# Autodesk Inventor assembly: hodoscopeHolder
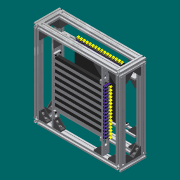
[picture p0: Inventor's stored thumbnail of the model, 180x180]
Saved by Autodesk Inventor 2016 (Build 200138000, 138)
## iProperties
Created: 2016-02-10
Part Number: hodoscopeHolder
Document SubType Name: Assembly
Designer: Sawaiz
Author: Sawaiz
## Documents named in this file (5)
- C:\Users\Sawaiz\OneDrive\projects\modularRICH\testMount\fingerHodoscope\hodoscopeHolder.iam
- C:\Users\Sawaiz\OneDrive\projects\modularRICH\testMount\fingerHodoscope\face.iam
- C:\Users\Sawaiz\OneDrive\projects\modularRICH\testMount\fingerHodoscope\hfs5-2020-HodoscopeSeperator.ipt
- C:\Users\Sawaiz\OneDrive\projects\modularRICH\testMount\frame\angleBracket.iam
- C:\Users\Sawaiz\OneDrive\projects\scintillatorPanel\4xStack.iam
## Components (24 placed, 4 different names)
1. face:1 [sub-assembly] — Flush:1, Flush:2, Symmetry:1, Symmetry:2, Symmetry:3, Flush:3, Flush:4, Flush:5, Flush:6, Mate:2, Mate:3, Flush:7, Flush:8, Flush:9, Flush:10, Flush:11, Flush:12, Flush:13, Flush:14, Flush:29, Mate:15, Mate:18, Mate:20, Flush:39, Mate:22, Mate:25, Flush:70, Mate:36, Flush:71, Mate:42
2. face:2 [sub-assembly] — Flush:1, Flush:2, Symmetry:1, Symmetry:2, Symmetry:3, Mate:1, Flush:15, Mate:23, Mate:26, Flush:53, Mate:34, Mate:37, Mate:38, Flush:72, Mate:45
3. hfs5-2020-HodoscopeSeperator:1 — Mate:1, Flush:3, Flush:12, Flush:13, Flush:14, Mate:35
4. hfs5-2020-HodoscopeSeperator:2 — Flush:4, Flush:9, Flush:10, Flush:11, Flush:15, Mate:27
5. hfs5-2020-HodoscopeSeperator:3 — Flush:6, Mate:2, Mate:3, Mate:39
6. hfs5-2020-HodoscopeSeperator:4 — Flush:5, Flush:7, Flush:8, Flush:38, Mate:24
7. angleBracket:1 [sub-assembly] — Flush:26, Mate:20, Flush:56
8. angleBracket:2 [sub-assembly] — Flush:26, Flush:27, Flush:30, Mate:15, Symmetry:6, Flush:56, Mate:40
9. angleBracket:3 [sub-assembly] — Flush:27, Flush:28, Flush:30, Symmetry:6, Flush:57, Mate:41
10. angleBracket:4 [sub-assembly] — Flush:28, Flush:29, Mate:18, Flush:57
11. angleBracket:5 [sub-assembly] — Flush:24, Flush:34, Flush:52, Flush:55, Mate:43
12. angleBracket:6 [sub-assembly] — Flush:23, Flush:24, Flush:32, Flush:50, Flush:51, Symmetry:4, Symmetry:5, Flush:54
13. angleBracket:7 [sub-assembly] — Flush:22, Flush:23, Flush:34, Flush:51, Flush:52, Symmetry:4, Flush:53, Mate:34, Flush:54, Mate:44
14. angleBracket:8 [sub-assembly] — Flush:22, Flush:32, Flush:50, Symmetry:5, Flush:55
15. angleBracket:9 [sub-assembly] — Flush:37, Flush:38, Flush:41, Mate:26, Mate:27
16. angleBracket:10 [sub-assembly] — Flush:36, Flush:37, Mate:22, Flush:40, Mate:24
17. angleBracket:11 [sub-assembly] — Flush:35, Flush:36, Flush:39, Mate:23, Flush:40
18. angleBracket:12 [sub-assembly] — Flush:35, Flush:41, Mate:25
19. 4xStack:1 [sub-assembly] — Mate:40, Mate:41, Flush:71, Mate:42
20. 4xStack:2 [sub-assembly] — Mate:43, Mate:44, Flush:72, Mate:45
21. angleBracket:13 [sub-assembly] — Flush:65, Flush:66, Flush:67, Flush:68, Mate:37
22. angleBracket:14 [sub-assembly] — Flush:63, Flush:64, Flush:68, Flush:69, Mate:39
23. angleBracket:15 [sub-assembly] — Flush:63, Flush:69, Mate:38
24. angleBracket:16 [sub-assembly] — Flush:64, Flush:65, Flush:66, Mate:35, Flush:67, Flush:70, Mate:36
## Relationships (85: Flush 55, Mate 24, Symmetry 6)
- Flush:1: face:1 ↔ face:2
- Flush:2: face:1 ↔ face:2
- Symmetry:1: face:1 ↔ face:2
- Symmetry:2: face:1 ↔ face:2
- Symmetry:3: face:1 ↔ face:2
- Mate:1: face:2 ↔ hfs5-2020-HodoscopeSeperator:1
- Flush:3: face:1 ↔ hfs5-2020-HodoscopeSeperator:1
- Flush:4: face:1 ↔ hfs5-2020-HodoscopeSeperator:2
- Flush:5: face:1 ↔ hfs5-2020-HodoscopeSeperator:4
- Flush:6: face:1 ↔ hfs5-2020-HodoscopeSeperator:3
- Mate:2: face:1 ↔ hfs5-2020-HodoscopeSeperator:3
- Mate:3: face:1 ↔ hfs5-2020-HodoscopeSeperator:3
- Flush:7: face:1 ↔ hfs5-2020-HodoscopeSeperator:4
- Flush:8: face:1 ↔ hfs5-2020-HodoscopeSeperator:4
- Flush:9: face:1 ↔ hfs5-2020-HodoscopeSeperator:2
- Flush:10: face:1 ↔ hfs5-2020-HodoscopeSeperator:2
- Flush:11: face:1 ↔ hfs5-2020-HodoscopeSeperator:2
- Flush:12: face:1 ↔ hfs5-2020-HodoscopeSeperator:1
- Flush:13: face:1 ↔ hfs5-2020-HodoscopeSeperator:1
- Flush:14: face:1 ↔ hfs5-2020-HodoscopeSeperator:1
- Flush:15: face:2 ↔ hfs5-2020-HodoscopeSeperator:2
- Flush:22: angleBracket:7 ↔ angleBracket:8
- Flush:23: angleBracket:6 ↔ angleBracket:7
- Flush:24: angleBracket:5 ↔ angleBracket:6
- Flush:26: angleBracket:1 ↔ angleBracket:2
- Flush:27: angleBracket:2 ↔ angleBracket:3
- Flush:28: angleBracket:3 ↔ angleBracket:4
- Flush:29: face:1 ↔ angleBracket:4
- Flush:30: angleBracket:2 ↔ angleBracket:3
- Mate:15: face:1 ↔ angleBracket:2
- Mate:18: face:1 ↔ angleBracket:4
- Mate:20: face:1 ↔ angleBracket:1
- Flush:32: angleBracket:6 ↔ angleBracket:8
- Flush:34: angleBracket:5 ↔ angleBracket:7
- Flush:35: angleBracket:11 ↔ angleBracket:12
- Flush:36: angleBracket:10 ↔ angleBracket:11
- Flush:37: angleBracket:9 ↔ angleBracket:10
- Flush:38: hfs5-2020-HodoscopeSeperator:4 ↔ angleBracket:9
- Flush:39: face:1 ↔ angleBracket:11
- Mate:22: face:1 ↔ angleBracket:10
- Mate:23: face:2 ↔ angleBracket:11
- Flush:40: angleBracket:10 ↔ angleBracket:11
- Mate:24: hfs5-2020-HodoscopeSeperator:4 ↔ angleBracket:10
- Flush:41: angleBracket:9 ↔ angleBracket:12
- Mate:25: face:1 ↔ angleBracket:12
- Mate:26: face:2 ↔ angleBracket:9
- Mate:27: hfs5-2020-HodoscopeSeperator:2 ↔ angleBracket:9
- Flush:50: angleBracket:6 ↔ angleBracket:8
- Flush:51: angleBracket:6 ↔ angleBracket:7
- Flush:52: angleBracket:5 ↔ angleBracket:7
- Symmetry:4: angleBracket:6 ↔ angleBracket:7
- Symmetry:5: angleBracket:6 ↔ angleBracket:8
- Symmetry:6: angleBracket:2 ↔ angleBracket:3
- Flush:53: face:2 ↔ angleBracket:7
- Mate:34: face:2 ↔ angleBracket:7
- Flush:54: angleBracket:6 ↔ angleBracket:7
- Flush:55: angleBracket:5 ↔ angleBracket:8
- Flush:56: angleBracket:1 ↔ angleBracket:2
- Flush:57: angleBracket:3 ↔ angleBracket:4
- [Flush]: angleBracket:15 ↔ angleBracket:16
- [Flush]: angleBracket:14 ↔ angleBracket:15
- [Flush]: angleBracket:13 ↔ angleBracket:14
- [Flush]: angleBracket:14 ↔ angleBracket:15
- [Flush]: angleBracket:13 ↔ angleBracket:16
- Flush:63: angleBracket:14 ↔ angleBracket:15
- Flush:64: angleBracket:14 ↔ angleBracket:16
- Flush:65: angleBracket:13 ↔ angleBracket:16
- Flush:66: angleBracket:13 ↔ angleBracket:16
- Mate:35: hfs5-2020-HodoscopeSeperator:1 ↔ angleBracket:16
- Flush:67: angleBracket:13 ↔ angleBracket:16
- Flush:68: angleBracket:13 ↔ angleBracket:14
- Flush:69: angleBracket:14 ↔ angleBracket:15
- Flush:70: face:1 ↔ angleBracket:16
- Mate:36: face:1 ↔ angleBracket:16
- Mate:37: face:2 ↔ angleBracket:13
- Mate:38: face:2 ↔ angleBracket:15
- Mate:39: hfs5-2020-HodoscopeSeperator:3 ↔ angleBracket:14
- Mate:40: angleBracket:2 ↔ 4xStack:1
- Mate:41: angleBracket:3 ↔ 4xStack:1
- Flush:71: face:1 ↔ 4xStack:1
- Mate:42: face:1 ↔ 4xStack:1
- Mate:43: angleBracket:5 ↔ 4xStack:2
- Mate:44: angleBracket:7 ↔ 4xStack:2
- Flush:72: face:2 ↔ 4xStack:2
- Mate:45: face:2 ↔ 4xStack:2
## Named parameters: d109_d55 = 0 mm, d110_d56 = 0 mm, d111_d57 = 0 mm, d112_d62 = 0 mm, d113_d64 = 0 mm
